# Autodesk Inventor assembly: escassembly
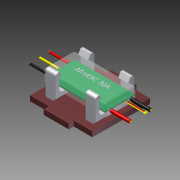
[picture p0: Inventor's stored thumbnail of the model, 180x180]
Saved by Autodesk Inventor 2012 (Build 160160000, 160)
## iProperties
Created: 2014-07-18
Part Number: escassembly
Document SubType Name: Assembly
Designer: Anon
Author: Anon
## Documents named in this file (4)
- D:\Dropbox\Courses\GP\git\dronestructure\electronics\afroesc\escassembly.iam
- D:\Dropbox\Courses\GP\git\dronestructure\electronics\afroesc\afroesc.iam
- D:\Dropbox\Courses\GP\git\dronestructure\electronics\afroesc\claw.ipt
- D:\Dropbox\Courses\GP\git\dronestructure\electronics\afroesc\escbase.ipt
## Components (4 placed, 3 different names)
1. afroesc:1 [sub-assembly] — Mate:7, Mate:8
2. claw:1 — Mate:4, Mate:5, Mate:6, Mate:7
3. claw:2 — Mate:1, Mate:2, Mate:3
4. escbase:1 — Mate:1, Mate:2, Mate:3, Mate:4, Mate:5, Mate:6, Mate:8
## Relationships (8: Mate 8)
- Mate:1: claw:2 ↔ escbase:1
- Mate:2: claw:2 ↔ escbase:1
- Mate:3: claw:2 ↔ escbase:1
- Mate:4: claw:1 ↔ escbase:1
- Mate:5: claw:1 ↔ escbase:1
- Mate:6: claw:1 ↔ escbase:1
- Mate:7: afroesc:1 ↔ claw:1
- Mate:8: afroesc:1 ↔ escbase:1
